# Autodesk Inventor assembly: втулка и звезда ура ура
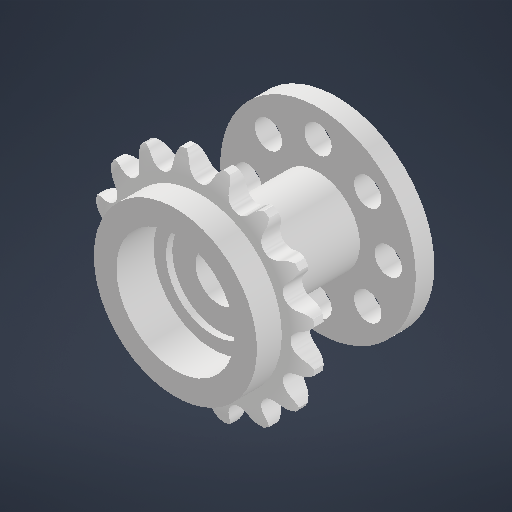
[picture p0: Inventor's stored thumbnail of the model, 512x512]
Saved by Autodesk Inventor 2025 (Build 290162000, 162)
## iProperties
Created: 2025-01-10
Part Number: втулка и звезда ура ура
Document SubType Name: Assembly
Designer: Phantom
Author: Phantom
## Documents named in this file (3)
- C:\Users\Phantom\Desktop\Phantom16950\втулка и звезда ура ура.iam
- C:\Users\Phantom\Desktop\Phantom16950\втулка для подш.ipt
- C:\Users\Phantom\Desktop\Phantom16950\Звездочка роликовой цепи22.ipt
## Components (2 placed, 2 different names)
1. втулка для подш:1 — Совмещение:1, Заподлицо:1
2. Звездочка роликовой цепи2:1 — Совмещение:1, Заподлицо:1
## Relationships (2: Mate 1, Flush 1)
- Совмещение:1 [Mate]: втулка для подш:1 ↔ Звездочка роликовой цепи2:1
- Заподлицо:1 [Flush] (4 mm): втулка для подш:1 ↔ Звездочка роликовой цепи2:1
